# Autodesk Inventor assembly: V5H2
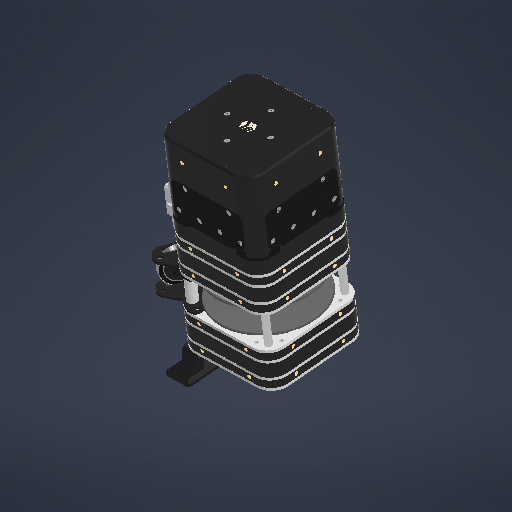
[picture p0: Inventor's stored thumbnail of the model, 512x512]
Saved by Autodesk Inventor 2026.1 (Build 301233000, 233)
## iProperties
Created: 2026-05-18
Part Number: V5H2
Document SubType Name: Assembly
Designer: aaron
Author: aaron
## Documents named in this file (25)
- D:\work\loopandpixel\openworkoutsystem\cad\v5\V5H2.iam
- D:\work\loopandpixel\openworkoutsystem\cad\v5\motor.iam
- D:\work\loopandpixel\openworkoutsystem\cad\v5\handle_metal.ipt
- D:\work\loopandpixel\openworkoutsystem\cad\v5\handle_insert.ipt
- D:\work\loopandpixel\openworkoutsystem\cad\v5\spool.iam
- D:\work\loopandpixel\openworkoutsystem\cad\v5\output_support.ipt
- D:\work\loopandpixel\openworkoutsystem\cad\v5\spool_spacer_driver.ipt
- D:\work\loopandpixel\openworkoutsystem\cad\v5\spool_spacer.ipt
- D:\work\loopandpixel\openworkoutsystem\cad\v5\M5x40mm_coupler.ipt
- D:\work\loopandpixel\openworkoutsystem\cad\v5\bearings\bearing_42x30x7.ipt
- D:\work\loopandpixel\openworkoutsystem\cad\v5\head_innter_top_42.ipt
- D:\work\loopandpixel\openworkoutsystem\cad\v5\bearings\bearing_12x8x8.ipt
- D:\work\loopandpixel\openworkoutsystem\cad\v5\moteus\20250427-moteus-x1-r1\20250427-moteus-x1-r1\20250427-moteus-x1-r1.ipt
- D:\work\loopandpixel\openworkoutsystem\cad\v5\20250328-x1-heat-spreader\20250328-x1-heat-spreader\20250328-x1-heat-spreader.ipt
- D:\work\loopandpixel\openworkoutsystem\cad\v5\mcthermal_plate.ipt
- D:\work\loopandpixel\openworkoutsystem\cad\v5\battery_pack_16s.ipt.iam
- D:\work\loopandpixel\openworkoutsystem\cad\v5\shaft_with_keyway.ipt
- D:\work\loopandpixel\openworkoutsystem\cad\v5\encoder_spacer.ipt
- D:\work\loopandpixel\openworkoutsystem\cad\v5\battery_spacer.ipt
- C:\Users\aaron\OneDrive\Documents\Inventor\Content Center Files\R2026\en-US\IS 6761\IS 6761 - M3 x 8 - 0.5.ipt
- D:\work\loopandpixel\openworkoutsystem\cad\v5\T-Display-S3-AMOLED-Touch-PCB-3D\T-Display-S3-AMOLED-Touch-PCB-3D\0-ALL_ASM_362_ASM_2_ASM.iam
- D:\work\loopandpixel\openworkoutsystem\cad\v5\button\button\button.ipt
- D:\work\loopandpixel\openworkoutsystem\cad\v5\encoder_magnet_holder.ipt
- D:\work\loopandpixel\openworkoutsystem\cad\v5\screen_top.ipt
- battery_pack_16s.ipt
## Components (51 placed, 23 different names)
1. motor:1 [sub-assembly] — Insert:1, Insert:2, Insert:5, Insert:6, Flush:1, Insert:12, Insert:13, Flush:12
2. handle_metal:1 — Insert:1, Insert:2, Insert:29, Flush:8
3. handle_insert:1 — Insert:29, Flush:8
4. motor:2 [sub-assembly] — Insert:7, Flush:1, Insert:14, Insert:15, Insert:17, Insert:18, Flush:2, Flush:3, Flush:6, Flush:7, Insert:31, Mate:33, Mate:34, Flush:13
5. spool:1 [sub-assembly] — Insert:10, Insert:11
6. output_support:1 — Insert:14, Insert:15, Insert:16, Insert:19, Tangent:1, Mate:31
7. output_support:2 — Insert:12, Insert:13, Mate:1
8. spool_spacer_driver:1 — Insert:7, Insert:8
9. spool_spacer_driver:2 — Insert:6, Mate:6
10. spool_spacer_driver:3 — Insert:5, Insert:9
11. spool_spacer:1 — Insert:9, Insert:10
12. spool_spacer:2 — Insert:8, Insert:11
13. M5x40mm_coupler:1 — Insert:16
14. M5x40mm_coupler:2 — Insert:19, Mate:2
15. M5x40mm_coupler:3 — Insert:18
16. M5x40mm_coupler:4 — Insert:17
17. bearing_42x30x7:1 — Insert:20, Mate:1
18. head_innter_top_42:1 — Insert:20, Tangent:1
19. bearing_12x8x8:1 — Mate:2, Insert:21, Mate:31
20. bearing_12x8x8:2 — Insert:21, Insert:22
21. bearing_12x8x8:3 — Insert:22, Insert:23
22. bearing_12x8x8:4 — Insert:23
23. 20250427-moteus-x1-r1:1
24. 20250328-x1-heat-spreader:1 — Insert:27, Insert:28
25. mcthermal_plate:1 — Flush:2, Flush:3, Flush:4, Flush:5, Insert:27, Insert:28, Mate:5, Mate:8, Mate:9, Mate:10, Mate:11, Mate:12, Mate:13, Mate:14, Mate:15, Mate:16, Mate:17, Mate:18, Mate:19, Mate:20, Mate:21, Mate:22, Mate:23, Mate:24, Mate:25, Mate:26, Mate:27, Mate:28, Mate:32
26. battery_pack_16s.ipt:1 [sub-assembly] — Flush:4, Flush:5, Mate:5, Flush:9, Mate:35
27. shaft_with_keyway:1 — Mate:6, Flush:12
28. encoder_spacer:1 — Flush:6, Flush:7, Mate:32, Mate:33
29. battery_spacer:1 — Mate:8, Mate:9, Mate:10, Flush:9, Insert:30
30. IS 6761 M3 x 8:1 — Mate:11
31. IS 6761 M3 x 8:2 — Mate:12
32. IS 6761 M3 x 8:3 — Mate:13
33. IS 6761 M3 x 8:4 — Mate:14
34. IS 6761 M3 x 8:5 — Mate:15
35. IS 6761 M3 x 8:6 — Mate:16
36. IS 6761 M3 x 8:7 — Mate:17
37. IS 6761 M3 x 8:8 — Mate:18
38. IS 6761 M3 x 8:9 — Mate:19
39. IS 6761 M3 x 8:10 — Mate:20
40. IS 6761 M3 x 8:11 — Mate:21
41. IS 6761 M3 x 8:12 — Mate:22
42. IS 6761 M3 x 8:13 — Mate:23
43. IS 6761 M3 x 8:14 — Mate:24
44. IS 6761 M3 x 8:15 — Mate:25
45. IS 6761 M3 x 8:16 — Mate:26
46. IS 6761 M3 x 8:17 — Mate:27
47. IS 6761 M3 x 8:18 — Mate:28
48. 0-ALL_ASM_362_ASM_2_ASM:1 [sub-assembly]
49. button:1 — Insert:30
50. encoder_magnet_holder:1 — Insert:31
51. screen_top:1 — Mate:34, Flush:13, Mate:35
## Relationships (71: Mate 31, Insert 28, Flush 11, Tangent 1)
- Insert:1: motor:1 ↔ handle_metal:1
- Insert:2: motor:1 ↔ handle_metal:1
- Insert:5: motor:1 ↔ spool_spacer_driver:3
- Insert:6: motor:1 ↔ spool_spacer_driver:2
- Insert:7: motor:2 ↔ spool_spacer_driver:1
- Insert:8: spool_spacer_driver:1 ↔ spool_spacer:2
- Insert:9: spool_spacer_driver:3 ↔ spool_spacer:1
- Insert:10: spool:1 ↔ spool_spacer:1
- Insert:11: spool:1 ↔ spool_spacer:2
- Flush:1: motor:1 ↔ motor:2
- Insert:12: motor:1 ↔ output_support:2
- Insert:13: motor:1 ↔ output_support:2
- Insert:14: motor:2 ↔ output_support:1
- Insert:15: motor:2 ↔ output_support:1
- Insert:16: output_support:1 ↔ M5x40mm_coupler:1
- Insert:17: motor:2 ↔ M5x40mm_coupler:4
- Insert:18: motor:2 ↔ M5x40mm_coupler:3
- Insert:19: output_support:1 ↔ M5x40mm_coupler:2
- Insert:20: bearing_42x30x7:1 ↔ head_innter_top_42:1
- Mate:1: output_support:2 ↔ bearing_42x30x7:1
- Mate:2: M5x40mm_coupler:2 ↔ bearing_12x8x8:1
- Insert:21: bearing_12x8x8:1 ↔ bearing_12x8x8:2
- Insert:22: bearing_12x8x8:2 ↔ bearing_12x8x8:3
- Insert:23: bearing_12x8x8:3 ↔ bearing_12x8x8:4
- [Insert]: 20250427-moteus-x1-r1:1 ↔ 20250328-x1-heat-spreader:1
- [Insert]: 20250427-moteus-x1-r1:1 ↔ 20250328-x1-heat-spreader:1
- [Mate]: 20250328-x1-heat-spreader:1 ↔ mcthermal_plate:1
- Flush:2: motor:2 ↔ mcthermal_plate:1
- Flush:3: motor:2 ↔ mcthermal_plate:1
- Flush:4: mcthermal_plate:1 ↔ battery_pack_16s.ipt:1
- Flush:5: mcthermal_plate:1 ↔ battery_pack_16s.ipt:1
- Insert:27: 20250328-x1-heat-spreader:1 ↔ mcthermal_plate:1
- Insert:28: 20250328-x1-heat-spreader:1 ↔ mcthermal_plate:1
- Mate:5 (0.1 mm): mcthermal_plate:1 ↔ battery_pack_16s.ipt:1
- Mate:6: spool_spacer_driver:2 ↔ shaft_with_keyway:1
- Flush:6: motor:2 ↔ encoder_spacer:1
- Flush:7: motor:2 ↔ encoder_spacer:1
- Tangent:1 (0.5 mm): output_support:1 ↔ head_innter_top_42:1
- Insert:29: handle_metal:1 ↔ handle_insert:1
- Flush:8: handle_metal:1 ↔ handle_insert:1
- Mate:8: mcthermal_plate:1 ↔ battery_spacer:1
- Mate:9: mcthermal_plate:1 ↔ battery_spacer:1
- Mate:10: mcthermal_plate:1 ↔ battery_spacer:1
- Flush:9: battery_pack_16s.ipt:1 ↔ battery_spacer:1
- Mate:11: mcthermal_plate:1 ↔ IS 6761 M3 x 8:1
- Mate:12: mcthermal_plate:1 ↔ IS 6761 M3 x 8:2
- Mate:13: mcthermal_plate:1 ↔ IS 6761 M3 x 8:3
- Mate:14: mcthermal_plate:1 ↔ IS 6761 M3 x 8:4
- Mate:15: mcthermal_plate:1 ↔ IS 6761 M3 x 8:5
- Mate:16: mcthermal_plate:1 ↔ IS 6761 M3 x 8:6
- Mate:17: mcthermal_plate:1 ↔ IS 6761 M3 x 8:7
- Mate:18: mcthermal_plate:1 ↔ IS 6761 M3 x 8:8
- Mate:19: mcthermal_plate:1 ↔ IS 6761 M3 x 8:9
- Mate:20: mcthermal_plate:1 ↔ IS 6761 M3 x 8:10
- Mate:21: mcthermal_plate:1 ↔ IS 6761 M3 x 8:11
- Mate:22: mcthermal_plate:1 ↔ IS 6761 M3 x 8:12
- Mate:23: mcthermal_plate:1 ↔ IS 6761 M3 x 8:13
- Mate:24: mcthermal_plate:1 ↔ IS 6761 M3 x 8:14
- Mate:25: mcthermal_plate:1 ↔ IS 6761 M3 x 8:15
- Mate:26: mcthermal_plate:1 ↔ IS 6761 M3 x 8:16
- Mate:27: mcthermal_plate:1 ↔ IS 6761 M3 x 8:17
- Mate:28: mcthermal_plate:1 ↔ IS 6761 M3 x 8:18
- Mate:31 (2 mm): output_support:1 ↔ bearing_12x8x8:1
- Flush:12 (-15 mm): motor:1 ↔ shaft_with_keyway:1
- Insert:30: battery_spacer:1 ↔ button:1
- Mate:32: mcthermal_plate:1 ↔ encoder_spacer:1
- Insert:31: motor:2 ↔ encoder_magnet_holder:1
- Mate:33: motor:2 ↔ encoder_spacer:1
- Mate:34: motor:2 ↔ screen_top:1
- Flush:13 (18 mm): motor:2 ↔ screen_top:1
- Mate:35: battery_pack_16s.ipt:1 ↔ screen_top:1
